# Autodesk Inventor assembly: Scanner
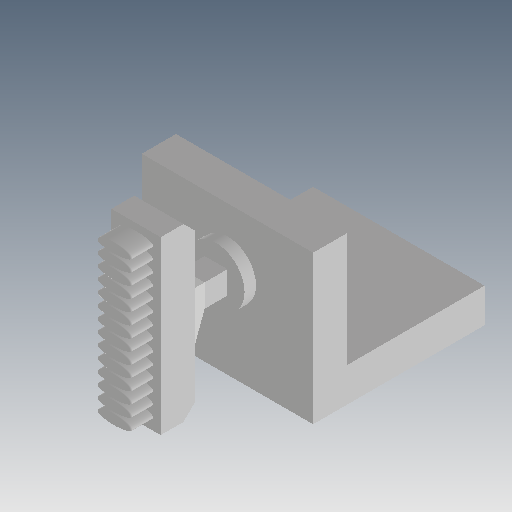
[picture p0: Inventor's stored thumbnail of the model, 512x512]
Saved by Autodesk Inventor 2020 (Build 240168000, 168)
## iProperties
Created: 2020-03-18
Part Number: Scanner
Document SubType Name: Assembly
Designer: franz
Author: franz
## Documents named in this file (3)
- E:\Privat\Projekte\SPS_Training\Unity_SPS_Simulation\Unity_SPS_Schrittkette\CAD\Foerderband_V1\Scanner\Scanner.iam
- E:\Privat\Projekte\SPS_Training\Unity_SPS_Simulation\Unity_SPS_Schrittkette\CAD\Foerderband_V1\Scanner\Staender.ipt
- E:\Privat\Projekte\SPS_Training\Unity_SPS_Simulation\Unity_SPS_Schrittkette\CAD\Foerderband_V1\Scanner\Scannerkopf.ipt
## Components (2 placed, 2 different names)
1. Staender:1 — Starr:1
2. Scannerkopf:1 — Starr:1
## Relationships (1: WeldJoint 1)
- Starr:1 [WeldJoint]: Staender:1 ↔ Scannerkopf:1
